# Autodesk Inventor assembly: Box_asm
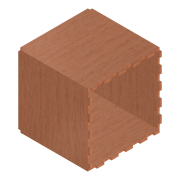
[picture p0: Inventor's stored thumbnail of the model, 180x180]
Saved by Autodesk Inventor 2022.1 (Build 261234000, 234)
## iProperties
Created: 2022-06-17
Part Number: Box_asm
Document SubType Name: Assembly
Designer: william
Author: william
## Documents named in this file (3)
- D:\Personal_Workspace\Cool Stuff\Stepper_Motor_Music\Resonant_Box\Box_asm.iam
- D:\Personal_Workspace\Cool Stuff\Stepper_Motor_Music\Resonant_Box\Base.ipt
- D:\Personal_Workspace\Cool Stuff\Stepper_Motor_Music\Resonant_Box\Top.ipt
## Components (5 placed, 2 different names)
1. Base:1 — Mate:1, Flush:1, Mate:2, Mate:3, Flush:2, Mate:4, Mate:5, Mate:7
2. Base:2 — Mate:5, Mate:6, Mate:7, Mate:8, Mate:9
3. Base:3 — Mate:3, Flush:2, Mate:4
4. Base:4 — Mate:1, Flush:1, Mate:2, Mate:6, Mate:10
5. Top:1 — Mate:8, Mate:9, Mate:10
## Relationships (12: Mate 10, Flush 2)
- Mate:1: Base:1 ↔ Base:4
- Flush:1: Base:1 ↔ Base:4
- Mate:2: Base:1 ↔ Base:4
- Mate:3: Base:1 ↔ Base:3
- Flush:2: Base:1 ↔ Base:3
- Mate:4: Base:1 ↔ Base:3
- Mate:5: Base:1 ↔ Base:2
- Mate:6: Base:2 ↔ Base:4
- Mate:7: Base:1 ↔ Base:2
- Mate:8: Base:2 ↔ Top:1
- Mate:9: Base:2 ↔ Top:1
- Mate:10: Base:4 ↔ Top:1
